# Autodesk Inventor assembly: handle
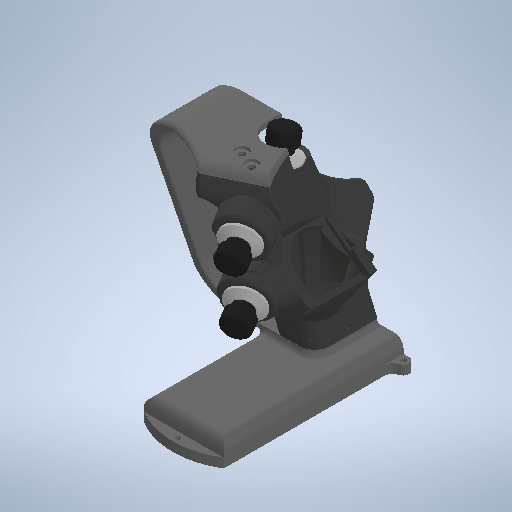
[picture p0: Inventor's stored thumbnail of the model, 512x512]
Saved by Autodesk Inventor 2026.1 (Build 301233020, 233B)
## iProperties
Created: 2026-01-22
Part Number: handle
Document SubType Name: Assembly
Designer: hibik
Author: hibik
## Documents named in this file (5)
- C:\Users\hibik\Documents\Robomech\HR\controller\hard\handle_right\handle.iam
- C:\Users\hibik\Documents\Robomech\HR\controller\hard\handle_right\handle_outside.ipt
- C:\Users\hibik\Documents\Robomech\HR\controller\hard\handle_right\pannel_push_sw.ipt
- C:\Users\hibik\Documents\Robomech\HR\controller\hard\handle_right\handle_inside.ipt
- C:\Users\hibik\Documents\Robomech\HR\controller\hard\handle_right\handle_monitor.ipt
## Components (6 placed, 4 different names)
1. handle_outside:1 — 挿入:1, 挿入:2, 挿入:3, フラッシュ:1, フラッシュ:2, フラッシュ:3, メイト:1, フラッシュ:4
2. pannel_push_sw:1 — 挿入:1
3. pannel_push_sw:2 — 挿入:2
4. pannel_push_sw:3 — 挿入:3
5. handle_inside:1 — フラッシュ:1, フラッシュ:2, フラッシュ:3, メイト:1, フラッシュ:4
6. handle_monitor:1 — フラッシュ:5, フラッシュ:6, フラッシュ:7
## Relationships (11: Flush 7, Insert 3, Mate 1)
- 挿入:1 [Insert]: handle_outside:1 ↔ pannel_push_sw:1
- 挿入:2 [Insert]: handle_outside:1 ↔ pannel_push_sw:2
- 挿入:3 [Insert]: handle_outside:1 ↔ pannel_push_sw:3
- フラッシュ:1 [Flush]: handle_outside:1 ↔ handle_inside:1
- フラッシュ:2 [Flush]: handle_outside:1 ↔ handle_inside:1
- フラッシュ:3 [Flush]: handle_outside:1 ↔ handle_inside:1
- メイト:1 [Mate]: handle_outside:1 ↔ handle_inside:1
- フラッシュ:4 [Flush]: handle_outside:1 ↔ handle_inside:1
- フラッシュ:5 [Flush]: handle_monitor:1
- フラッシュ:6 [Flush]: handle_monitor:1
- フラッシュ:7 [Flush]: handle_monitor:1
